# Autodesk Inventor assembly: RT_FRM_A_003_FrameV5
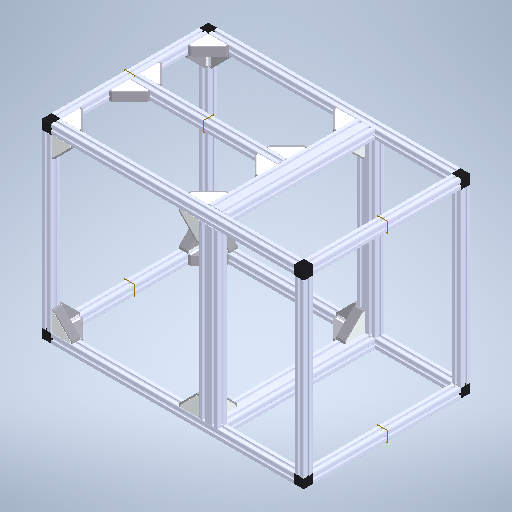
[picture p0: Inventor's stored thumbnail of the model, 512x512]
Saved by Autodesk Inventor 2025.4 (Build 294407000, 407)
## iProperties
Created: 2026-07-28
Part Number: RT_FRM_A_003_FrameV5
Document SubType Name: Assembly
Designer: louis
Mass: 29324.3 g
Surface Area: 138303 cm^2
Volume: 15957.5 cm^3
Density: 1.83764 g/cm^3
Author: louis
## Documents named in this file (15)
- C:\Users\louis\OneDrive\Desktop\R_Trident\02_CAD\04_Subassemblies\RT_FRM_A_003_FrameV5.iam
- C:\Users\louis\OneDrive\Desktop\R_Trident\02_CAD\01_Standard_Parts\03_FRM_Fastener\3Way-40.ipt
- C:\Users\louis\OneDrive\Desktop\R_Trident\02_CAD\01_Standard_Parts\02_FRM_Extrusions_Frame_V5\4040x920.ipt
- C:\Users\louis\OneDrive\Desktop\R_Trident\02_CAD\01_Standard_Parts\02_FRM_Extrusions_Frame_V5\4040x620.ipt
- C:\Users\louis\OneDrive\Desktop\R_Trident\02_CAD\01_Standard_Parts\02_FRM_Extrusions_Frame_V5\4080x620.ipt
- C:\Users\louis\OneDrive\Desktop\R_Trident\02_CAD\01_Standard_Parts\02_FRM_Extrusions_Frame_V5\4080x720.ipt
- C:\Users\louis\OneDrive\Desktop\R_Trident\02_CAD\01_Standard_Parts\02_FRM_Extrusions_Frame_V5\4040x720.ipt
- C:\Users\louis\OneDrive\Desktop\R_Trident\02_CAD\01_Standard_Parts\03_FRM_Fastener\3Way-40_cover.ipt
- C:\Users\louis\OneDrive\Desktop\R_Trident\02_CAD\03_Parts_Custom\RT_FRM_V5_MC_01_DynamicsBottom.ipt
- C:\Users\louis\OneDrive\Desktop\R_Trident\02_CAD\03_Parts_Custom\RT_FRM_V5_MC_01_DynamicsRear.ipt
- C:\Users\louis\OneDrive\Desktop\R_Trident\02_CAD\03_Parts_Custom\RT_FRM_V5_MC_01_DynamicsTop.ipt
- C:\Users\louis\OneDrive\Desktop\R_Trident\02_CAD\03_Parts_Custom\RT_FRM_V5_MC_01_DynamicsLeft.ipt
- C:\Users\louis\OneDrive\Desktop\R_Trident\02_CAD\03_Parts_Custom\RT_FRM_V5_MC_01_ElectronicsRight.ipt
- C:\Users\louis\OneDrive\Desktop\R_Trident\02_CAD\03_Parts_Custom\RT_FRM_V5_MC_01_ElectronicsBottom.ipt
- C:\Users\louis\OneDrive\Desktop\R_Trident\02_CAD\01_Standard_Parts\03_FRM_Fastener\4080L\A_4080L.iam
## Components (67 placed, 14 different names)
1. 3Way-40:1 — Mate:1, Mate:2, Flush:1, Mate:3, Mate:5, Mate:10, Mate:17, Mate:18, Mate:41, Mate:43, Mate:47, Mate:49, Flush:32, Flush:33, Flush:34
2. 3Way-40:2 — Mate:3, Mate:4, Mate:8, Mate:23, Mate:25, Mate:40, Mate:48, Flush:29, Flush:30, Flush:31
3. 3Way-40:3 — Mate:4, Mate:6, Mate:7, Mate:20, Mate:21, Mate:38, Mate:39, Mate:45, Flush:38, Flush:39, Flush:40
4. 3Way-40:4 — Mate:5, Mate:6, Mate:12, Mate:16, Mate:42, Mate:44, Mate:46, Flush:35, Flush:36, Flush:37
5. 3Way-40:5 — Mate:7, Mate:9, Mate:13, Mate:22, Mate:30, Mate:34, Flush:47, Flush:48, Flush:49
6. 3Way-40:6 — Mate:8, Mate:9, Mate:11, Mate:24, Mate:32, Mate:33, Mate:37, Flush:41, Flush:42, Flush:43
7. 3Way-40:7 — Mate:10, Mate:11, Mate:19, Mate:26, Mate:27, Mate:35, Mate:36, Flush:50, Flush:51, Flush:52
8. 3Way-40:8 — Mate:12, Mate:13, Mate:14, Mate:15, Mate:28, Mate:29, Mate:31, Flush:44, Flush:45, Flush:46
9. 4040x920:1 — Mate:14, Mate:15, Mate:16, Flush:2, Mate:53, Flush:6, Flush:19, Flush:21, Flush:92, Flush:93, Flush:94, Flush:95, Mate:115, Mate:117, Mate:119, Mate:120, Mate:121, Mate:122, Mate:124, Mate:129
10. 4040x920:2 — Mate:17, Mate:18, Mate:19, Flush:5, Mate:50, Mate:52, Flush:8, Flush:17, Flush:18, Mate:83, Mate:86, Mate:111, Mate:113
11. 4040x920:3 — Mate:20, Mate:21, Mate:22, Flush:3, Mate:107, Mate:110, Mate:125, Mate:127
12. 4040x920:4 — Mate:23, Mate:24, Mate:25, Flush:4, Mate:51, Flush:11, Flush:12, Flush:13, Flush:14, Flush:54, Flush:84, Flush:85, Flush:86, Flush:87, Mate:88, Mate:90, Mate:99, Mate:100, Mate:101, Mate:102, Mate:103, Mate:106, Mate:136
13. 4040x620:1 — Mate:26, Mate:27, Mate:28, Flush:16, Flush:18, Flush:19, Flush:20, Flush:53, Mate:94, Mate:98, Mate:112, Mate:118
14. 4040x720:3 — Mate:35, Mate:36, Mate:37, Flush:14, Flush:15, Flush:16, Flush:17, Flush:56, Mate:84, Mate:89, Mate:91, Mate:93
15. 4040x620:3 — Mate:32, Mate:33, Mate:34, Flush:13, Flush:15, Mate:54, Flush:88, Flush:89, Flush:90, Flush:91, Mate:92, Mate:96, Mate:105, Mate:108, Mate:144, Mate:148
16. 4040x720:1 — Mate:29, Mate:30, Mate:31, Flush:20, Flush:21, Mate:95, Mate:97, Mate:128, Mate:130
17. 4040x620:5 — Mate:38, Mate:39, Mate:40, Flush:10, Flush:12, Flush:57
18. 4040x620:6 — Mate:41, Mate:42, Mate:43, Flush:6, Flush:7, Flush:8, Flush:9, Flush:58
19. 4040x720:4 — Mate:44, Mate:45, Mate:46, Flush:7
20. 4040x720:2 — Mate:47, Mate:48, Mate:49, Flush:9, Flush:10, Flush:11
21. 4080x620:1 — Flush:3, Mate:51, Flush:22, Flush:24, Mate:54, Flush:55, Mate:79, Mate:82, Mate:104, Mate:109, Mate:135, Flush:98, Mate:142, Mate:145
22. 4080x720:2 — Flush:2, Mate:53, Flush:24, Mate:56, Mate:77, Mate:80, Mate:123, Mate:126, Symmetry:2
23. 4080x620:3 — Flush:5, Mate:52, Flush:23, Mate:75, Mate:78, Mate:114, Mate:116
24. 4080x720:1 — Flush:4, Mate:50, Flush:22, Flush:23, Mate:55, Mate:76, Mate:81, Mate:85, Mate:87, Symmetry:2
25. 3Way-40_cover:1 — Flush:29, Flush:30, Flush:31
26. 3Way-40_cover:2 — Flush:32, Flush:33, Flush:34
27. 3Way-40_cover:3 — Flush:35, Flush:36, Flush:37
28. 3Way-40_cover:4 — Flush:38, Flush:39, Flush:40
29. 3Way-40_cover:5 — Flush:41, Flush:42, Flush:43
30. 3Way-40_cover:6 — Flush:47, Flush:48, Flush:49
31. 3Way-40_cover:7 — Flush:50, Flush:51, Flush:52
32. 3Way-40_cover:8 — Flush:44, Flush:45, Flush:46
33. RT_FRM_V5_MC_01_DynamicsBottom:1 — Flush:53
34. RT_FRM_V5_MC_01_DynamicsRear:1 — Flush:54
35. RT_FRM_V5_MC_01_DynamicsTop:1 — Flush:55
36. RT_FRM_V5_MC_01_DynamicsLeft:1 — Flush:56
37. RT_FRM_V5_MC_01_ElectronicsRight:1 — Flush:57
38. RT_FRM_V5_MC_01_ElectronicsBottom:1 — Flush:58
39. A_4080L:1 [sub-assembly] — Mate:71, Mate:77, Mate:78
40. A_4080L:2 [sub-assembly] — Flush:84, Mate:83, Mate:84
41. A_4080L:3 [sub-assembly] — Flush:85, Mate:85, Mate:86
42. A_4080L:4 [sub-assembly] — Flush:86, Mate:89, Mate:90
43. A_4080L:5 [sub-assembly] — Mate:72, Mate:81, Mate:82
44. A_4080L:6 [sub-assembly] — Mate:73, Mate:79, Mate:80
45. A_4080L:7 [sub-assembly] — Mate:74, Mate:75, Mate:76
46. A_4080L:8 [sub-assembly] — Flush:87, Mate:87, Mate:88
47. A_4080L:9 [sub-assembly] — Flush:88, Mate:91, Mate:92
48. A_4080L:10 [sub-assembly] — Flush:89, Mate:95, Mate:96
49. A_4080L:11 [sub-assembly] — Flush:90, Mate:97, Mate:98
50. A_4080L:12 [sub-assembly] — Flush:91, Mate:93, Mate:94
51. A_4080L:13 [sub-assembly] — Mate:99, Mate:105, Mate:106
52. A_4080L:14 [sub-assembly] — Mate:100, Mate:109, Mate:110
53. A_4080L:15 [sub-assembly] — Mate:101, Mate:107, Mate:108
54. A_4080L:16 [sub-assembly] — Mate:102, Mate:103, Mate:104
55. A_4080L:17 [sub-assembly] — Flush:92, Mate:117, Mate:118
56. A_4080L:18 [sub-assembly] — Flush:93, Mate:113, Mate:114
57. A_4080L:19 [sub-assembly] — Flush:94, Mate:115, Mate:116
58. A_4080L:20 [sub-assembly] — Flush:95, Mate:111, Mate:112
59. A_4080L:21 [sub-assembly] — Mate:119, Mate:125, Mate:126
60. A_4080L:22 [sub-assembly] — Mate:120, Mate:129, Mate:130
61. A_4080L:23 [sub-assembly] — Mate:121, Mate:127, Mate:128
62. A_4080L:24 [sub-assembly] — Mate:122, Mate:123, Mate:124
63. 4040x620:7 — Mate:135, Flush:98, Mate:136, Mate:137, Mate:138, Mate:139, Mate:140, Mate:141, Mate:143, Mate:146, Mate:147
64. A_4080L:25 [sub-assembly] — Mate:138, Mate:147, Mate:148
65. A_4080L:26 [sub-assembly] — Mate:139, Mate:145, Mate:146
66. A_4080L:27 [sub-assembly] — Mate:137, Mate:143, Mate:144
67. A_4080L:28 [sub-assembly] — Mate:140, Mate:141, Mate:142
## Relationships (201: Mate 133, Flush 67, Symmetry 1)
- Mate:1: 3Way-40:1
- Mate:2: 3Way-40:1
- Flush:1: 3Way-40:1
- Mate:3: 3Way-40:1 ↔ 3Way-40:2
- Mate:4: 3Way-40:2 ↔ 3Way-40:3
- Mate:5: 3Way-40:1 ↔ 3Way-40:4
- Mate:6: 3Way-40:3 ↔ 3Way-40:4
- Mate:7: 3Way-40:3 ↔ 3Way-40:5
- Mate:8: 3Way-40:2 ↔ 3Way-40:6
- Mate:9: 3Way-40:5 ↔ 3Way-40:6
- Mate:10: 3Way-40:1 ↔ 3Way-40:7
- Mate:11: 3Way-40:6 ↔ 3Way-40:7
- Mate:12: 3Way-40:4 ↔ 3Way-40:8
- Mate:13: 3Way-40:5 ↔ 3Way-40:8
- Mate:14: 3Way-40:8 ↔ 4040x920:1
- Mate:15: 3Way-40:8 ↔ 4040x920:1
- Mate:16: 3Way-40:4 ↔ 4040x920:1
- Mate:17: 3Way-40:1 ↔ 4040x920:2
- Mate:18: 3Way-40:1 ↔ 4040x920:2
- Mate:19: 3Way-40:7 ↔ 4040x920:2
- Mate:20: 3Way-40:3 ↔ 4040x920:3
- Mate:21: 3Way-40:3 ↔ 4040x920:3
- Mate:22: 3Way-40:5 ↔ 4040x920:3
- Mate:23: 3Way-40:2 ↔ 4040x920:4
- Mate:24: 3Way-40:6 ↔ 4040x920:4
- Mate:25: 3Way-40:2 ↔ 4040x920:4
- Mate:26: 3Way-40:7 ↔ 4040x620:1
- Mate:27: 3Way-40:7 ↔ 4040x620:1
- Mate:28: 3Way-40:8 ↔ 4040x620:1
- Mate:29: 3Way-40:8 ↔ 4040x720:1
- Mate:30: 3Way-40:5 ↔ 4040x720:1
- Mate:31: 3Way-40:8 ↔ 4040x720:1
- Mate:32: 3Way-40:6 ↔ 4040x620:3
- Mate:33: 3Way-40:6 ↔ 4040x620:3
- Mate:34: 3Way-40:5 ↔ 4040x620:3
- Mate:35: 3Way-40:7 ↔ 4040x720:3
- Mate:36: 3Way-40:7 ↔ 4040x720:3
- Mate:37: 3Way-40:6 ↔ 4040x720:3
- Mate:38: 3Way-40:3 ↔ 4040x620:5
- Mate:39: 3Way-40:3 ↔ 4040x620:5
- Mate:40: 3Way-40:2 ↔ 4040x620:5
- Mate:41: 3Way-40:1 ↔ 4040x620:6
- Mate:42: 3Way-40:4 ↔ 4040x620:6
- Mate:43: 3Way-40:1 ↔ 4040x620:6
- Mate:44: 3Way-40:4 ↔ 4040x720:4
- Mate:45: 3Way-40:3 ↔ 4040x720:4
- Mate:46: 3Way-40:4 ↔ 4040x720:4
- Mate:47: 3Way-40:1 ↔ 4040x720:2
- Mate:48: 3Way-40:2 ↔ 4040x720:2
- Mate:49: 3Way-40:1 ↔ 4040x720:2
- Flush:2: 4040x920:1 ↔ 4080x720:2
- Flush:3: 4040x920:3 ↔ 4080x620:1
- Flush:4: 4040x920:4 ↔ 4080x720:1
- Flush:5: 4040x920:2 ↔ 4080x620:3
- Mate:50: 4040x920:2 ↔ 4080x720:1
- Mate:51: 4040x920:4 ↔ 4080x620:1
- Mate:52: 4040x920:2 ↔ 4080x620:3
- Mate:53: 4040x920:1 ↔ 4080x720:2
- Flush:6: 4040x920:1 ↔ 4040x620:6
- Flush:7: 4040x620:6 ↔ 4040x720:4
- Flush:8: 4040x920:2 ↔ 4040x620:6
- Flush:9: 4040x620:6 ↔ 4040x720:2
- Flush:10: 4040x620:5 ↔ 4040x720:2
- Flush:11: 4040x920:4 ↔ 4040x720:2
- Flush:12: 4040x920:4 ↔ 4040x620:5
- Flush:13: 4040x920:4 ↔ 4040x620:3
- Flush:14: 4040x920:4 ↔ 4040x720:3
- Flush:15: 4040x720:3 ↔ 4040x620:3
- Flush:16: 4040x620:1 ↔ 4040x720:3
- Flush:17: 4040x920:2 ↔ 4040x720:3
- Flush:18: 4040x920:2 ↔ 4040x620:1
- Flush:19: 4040x920:1 ↔ 4040x620:1
- Flush:20: 4040x620:1 ↔ 4040x720:1
- Flush:21: 4040x920:1 ↔ 4040x720:1
- Flush:22: 4080x620:1 ↔ 4080x720:1
- Flush:23: 4080x620:3 ↔ 4080x720:1
- Flush:24: 4080x620:1 ↔ 4080x720:2
- Mate:54 (620 mm): 4040x620:3 ↔ 4080x620:1
- Mate:55: 4080x720:1
- Mate:56: 4080x720:2
- Mate:57
- Mate:58
- Flush:29: 3Way-40:2 ↔ 3Way-40_cover:1
- Flush:30: 3Way-40:2 ↔ 3Way-40_cover:1
- Flush:31: 3Way-40:2 ↔ 3Way-40_cover:1
- Flush:32: 3Way-40:1 ↔ 3Way-40_cover:2
- Flush:33: 3Way-40:1 ↔ 3Way-40_cover:2
- Flush:34: 3Way-40:1 ↔ 3Way-40_cover:2
- Flush:35: 3Way-40:4 ↔ 3Way-40_cover:3
- Flush:36: 3Way-40:4 ↔ 3Way-40_cover:3
- Flush:37: 3Way-40:4 ↔ 3Way-40_cover:3
- Flush:38: 3Way-40:3 ↔ 3Way-40_cover:4
- Flush:39: 3Way-40:3 ↔ 3Way-40_cover:4
- Flush:40: 3Way-40:3 ↔ 3Way-40_cover:4
- Flush:41: 3Way-40:6 ↔ 3Way-40_cover:5
- Flush:42: 3Way-40:6 ↔ 3Way-40_cover:5
- Flush:43: 3Way-40:6 ↔ 3Way-40_cover:5
- Flush:44: 3Way-40:8 ↔ 3Way-40_cover:8
- Flush:45: 3Way-40:8 ↔ 3Way-40_cover:8
- Flush:46: 3Way-40:8 ↔ 3Way-40_cover:8
- Flush:47: 3Way-40:5 ↔ 3Way-40_cover:6
- Flush:48: 3Way-40:5 ↔ 3Way-40_cover:6
- Flush:49: 3Way-40:5 ↔ 3Way-40_cover:6
- Flush:50: 3Way-40:7 ↔ 3Way-40_cover:7
- Flush:51: 3Way-40:7 ↔ 3Way-40_cover:7
- Flush:52: 3Way-40:7 ↔ 3Way-40_cover:7
- Flush:53: 4040x620:1 ↔ RT_FRM_V5_MC_01_DynamicsBottom:1
- Flush:54: 4040x920:4 ↔ RT_FRM_V5_MC_01_DynamicsRear:1
- Flush:55: 4080x620:1 ↔ RT_FRM_V5_MC_01_DynamicsTop:1
- Flush:56: 4040x720:3 ↔ RT_FRM_V5_MC_01_DynamicsLeft:1
- Flush:57: 4040x620:5 ↔ RT_FRM_V5_MC_01_ElectronicsRight:1
- Flush:58: 4040x620:6 ↔ RT_FRM_V5_MC_01_ElectronicsBottom:1
- Mate:71 (-40 mm): A_4080L:1
- Mate:72 (-40 mm): A_4080L:5
- Mate:73 (-40 mm): A_4080L:6
- Mate:74 (-40 mm): A_4080L:7
- Mate:75: 4080x620:3 ↔ A_4080L:7
- Mate:76: 4080x720:1 ↔ A_4080L:7
- Mate:77: 4080x720:2 ↔ A_4080L:1
- Mate:78: 4080x620:3 ↔ A_4080L:1
- Mate:79: 4080x620:1 ↔ A_4080L:6
- Mate:80: 4080x720:2 ↔ A_4080L:6
- Mate:81: 4080x720:1 ↔ A_4080L:5
- Mate:82: 4080x620:1 ↔ A_4080L:5
- Flush:84: 4040x920:4 ↔ A_4080L:2
- Flush:85: 4040x920:4 ↔ A_4080L:3
- Flush:86: 4040x920:4 ↔ A_4080L:4
- Flush:87: 4040x920:4 ↔ A_4080L:8
- Mate:83: 4040x920:2 ↔ A_4080L:2
- Mate:84: 4040x720:3 ↔ A_4080L:2
- Mate:85: 4080x720:1 ↔ A_4080L:3
- Mate:86: 4040x920:2 ↔ A_4080L:3
- Mate:87: 4080x720:1 ↔ A_4080L:8
- Mate:88: 4040x920:4 ↔ A_4080L:8
- Mate:89: 4040x720:3 ↔ A_4080L:4
- Mate:90: 4040x920:4 ↔ A_4080L:4
- Flush:88: 4040x620:3 ↔ A_4080L:9
- Flush:89: 4040x620:3 ↔ A_4080L:10
- Flush:90: 4040x620:3 ↔ A_4080L:11
- Flush:91: 4040x620:3 ↔ A_4080L:12
- Mate:91: 4040x720:3 ↔ A_4080L:9
- Mate:92: 4040x620:3 ↔ A_4080L:9
- Mate:93: 4040x720:3 ↔ A_4080L:12
- Mate:94: 4040x620:1 ↔ A_4080L:12
- Mate:95: 4040x720:1 ↔ A_4080L:10
- Mate:96: 4040x620:3 ↔ A_4080L:10
- Mate:97: 4040x720:1 ↔ A_4080L:11
- Mate:98: 4040x620:1 ↔ A_4080L:11
- Mate:99: 4040x920:4 ↔ A_4080L:13
- Mate:100: 4040x920:4 ↔ A_4080L:14
- Mate:101: 4040x920:4 ↔ A_4080L:15
- Mate:102: 4040x920:4 ↔ A_4080L:16
- Mate:103: 4040x920:4 ↔ A_4080L:16
- Mate:104: 4080x620:1 ↔ A_4080L:16
- Mate:105: 4040x620:3 ↔ A_4080L:13
- Mate:106: 4040x920:4 ↔ A_4080L:13
- Mate:107: 4040x920:3 ↔ A_4080L:15
- Mate:108: 4040x620:3 ↔ A_4080L:15
- Mate:109: 4080x620:1 ↔ A_4080L:14
- Mate:110: 4040x920:3 ↔ A_4080L:14
- Flush:92: 4040x920:1 ↔ A_4080L:17
- Flush:93: 4040x920:1 ↔ A_4080L:18
- Flush:94: 4040x920:1 ↔ A_4080L:19
- Flush:95: 4040x920:1 ↔ A_4080L:20
- Mate:111: 4040x920:2 ↔ A_4080L:20
- Mate:112: 4040x620:1 ↔ A_4080L:20
- Mate:113: 4040x920:2 ↔ A_4080L:18
- Mate:114: 4080x620:3 ↔ A_4080L:18
- Mate:115: 4040x920:1 ↔ A_4080L:19
- Mate:116: 4080x620:3 ↔ A_4080L:19
- Mate:117: 4040x920:1 ↔ A_4080L:17
- Mate:118: 4040x620:1 ↔ A_4080L:17
- Mate:119: 4040x920:1 ↔ A_4080L:21
- Mate:120: 4040x920:1 ↔ A_4080L:22
- Mate:121: 4040x920:1 ↔ A_4080L:23
- Mate:122: 4040x920:1 ↔ A_4080L:24
- Mate:123: 4080x720:2 ↔ A_4080L:24
- Mate:124: 4040x920:1 ↔ A_4080L:24
- Mate:125: 4040x920:3 ↔ A_4080L:21
- Mate:126: 4080x720:2 ↔ A_4080L:21
- Mate:127: 4040x920:3 ↔ A_4080L:23
- Mate:128: 4040x720:1 ↔ A_4080L:23
- Mate:129: 4040x920:1 ↔ A_4080L:22
- Mate:130: 4040x720:1 ↔ A_4080L:22
- Symmetry:2: 4080x720:2 ↔ 4080x720:1
- Mate:134
- Mate:135: 4080x620:1 ↔ 4040x620:7
- Flush:98: 4080x620:1 ↔ 4040x620:7
- Mate:136 (290 mm): 4040x920:4 ↔ 4040x620:7
- Mate:137: 4040x620:7 ↔ A_4080L:27
- Mate:138: 4040x620:7 ↔ A_4080L:25
- Mate:139: 4040x620:7 ↔ A_4080L:26
- Mate:140: 4040x620:7 ↔ A_4080L:28
- Mate:141: 4040x620:7 ↔ A_4080L:28
- Mate:142: 4080x620:1 ↔ A_4080L:28
- Mate:143: 4040x620:7 ↔ A_4080L:27
- Mate:144: 4040x620:3 ↔ A_4080L:27
- Mate:145: 4080x620:1 ↔ A_4080L:26
- Mate:146: 4040x620:7 ↔ A_4080L:26
- Mate:147: 4040x620:7 ↔ A_4080L:25
- Mate:148: 4040x620:3 ↔ A_4080L:25
